# Autodesk Inventor assembly: linearActuatorWithPvcArm
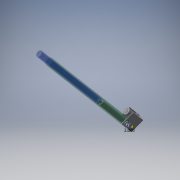
[picture p0: Inventor's stored thumbnail of the model, 180x180]
Saved by Autodesk Inventor 2018.2 (Build 222227000, 227)
## iProperties
Created: 2017-04-29
Part Number: linearActuatorWithPvcArm
Document SubType Name: Assembly
Designer: steele
Mass: 2624.32 g
Surface Area: 8704.67 cm^2
Volume: 2178.65 cm^3
Density: 1.20456 g/cm^3
Author: steele
## Documents named in this file (9)
- D:\snobotics\CAD-Development\robSteele\2018-FRC\GripperArm\linearActuatorWithPvcArm.iam
- D:\snobotics\CAD-Development\robSteele\SnoBotics2017\Arm\am-0077a-500 Key Hub r2.ipt
- D:\snobotics\CAD-Development\robSteele\SnoBotics2017\Arm\robotArmWithWormGearBox\Design Accelerator\Bolted Connection1.iam
- D:\snobotics\CAD-MfgResources\Andy-Mark\Linear Actuators\DART 12 in Actuator AM-3072a\am-3072aDART12.iam
- D:\snobotics\CAD-Development\robSteele\2018-FRC\GripperArm\supportPlateForLinearActuator.ipt
- D:\snobotics\CAD-Development\robSteele\2018-FRC\PVC Pipe\2_5-inch schedule 40 forArm.ipt
- D:\snobotics\CAD-Development\robSteele\SnoBotics2017\Arm\am-0077a-500 Key Hub r2_MIR1.ipt
- D:\snobotics\CAD-Development\robSteele\2018-FRC\GripperArm\supportPlateForLinearActuator_MIR1.ipt
- D:\snobotics\CAD-Development\robSteele\2018-FRC\PVC Pipe\2_0-inch schedule 40 for Arm.ipt
## Components (8 placed, 8 different names)
1. am-0077a-500 Key Hub r2:1 — Insert:8, Insert:9, Flush:3
2. Bolted Connection:1 [sub-assembly]
3. am-3072aDART12:1 [sub-assembly] — Mate:6, Flush:1, Flush:2, Insert:12, Insert:15
4. supportPlateForLinearActuator:1 — Insert:8, Insert:9, Mate:6, Flush:1, Flush:2
5. 2_5-inch schedule 40 forArm:1 — Insert:12
6. am-0077a-500 Key Hub r2_MIR1:1 — Insert:13, Insert:14, Mate:7
7. supportPlateForLinearActuator_MIR1:1 — Insert:13, Insert:14
8. 2_0-inch schedule 40 for Arm:1 — Insert:15
## Relationships (11: Insert 6, Flush 3, Mate 2)
- Insert:8: am-0077a-500 Key Hub r2:1 ↔ supportPlateForLinearActuator:1
- Insert:9: am-0077a-500 Key Hub r2:1 ↔ supportPlateForLinearActuator:1
- Mate:6: am-3072aDART12:1 ↔ supportPlateForLinearActuator:1
- Flush:1: am-3072aDART12:1 ↔ supportPlateForLinearActuator:1
- Flush:2: am-3072aDART12:1 ↔ supportPlateForLinearActuator:1
- Flush:3 (34.925 mm): am-0077a-500 Key Hub r2:1
- Insert:12 (-381 mm): am-3072aDART12:1 ↔ 2_5-inch schedule 40 forArm:1
- Insert:13: am-0077a-500 Key Hub r2_MIR1:1 ↔ supportPlateForLinearActuator_MIR1:1
- Insert:14: am-0077a-500 Key Hub r2_MIR1:1 ↔ supportPlateForLinearActuator_MIR1:1
- Mate:7 (47.625 mm): am-0077a-500 Key Hub r2_MIR1:1
- Insert:15: am-3072aDART12:1 ↔ 2_0-inch schedule 40 for Arm:1
